# Autodesk Inventor assembly: PanelMountNew Sliced
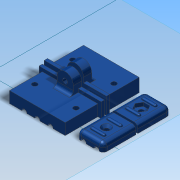
[picture p0: Inventor's stored thumbnail of the model, 180x180]
Saved by Autodesk Inventor 2014 SP2 (Build 180246200, 246)
## iProperties
Created: 2014-06-07
Part Number: PanelMountNew Sliced
Document SubType Name: Assembly
Designer: dliu
Author: dliu
## Documents named in this file (8)
- C:\Users\dliu\Dropbox\dbhome\electric-longboard\dliu\PanelMountNew Sliced.iam
- C:\Users\dliu\Dropbox\dbhome\electric-longboard\dliu\Electronics\Solid2.ipt
- C:\Users\dliu\Dropbox\dbhome\electric-longboard\dliu\Electronics\Solid3.ipt
- C:\Users\dliu\Dropbox\dbhome\electric-longboard\dliu\Electronics\Solid4.ipt
- C:\Users\dliu\Dropbox\dbhome\electric-longboard\dliu\Electronics\Solid5.ipt
- C:\Users\dliu\Dropbox\dbhome\electric-longboard\dliu\Electronics\Solid6.ipt
- C:\Users\dliu\Dropbox\dbhome\electric-longboard\dliu\Electronics\Solid7.ipt
- C:\Users\dliu\Dropbox\dbhome\electric-longboard\dliu\Electronics\Key.iam
## Components (7 placed, 7 different names)
1. Solid2:1 — Mate:5
2. Solid3:1 — Mate:4
3. Solid4:1 — Mate:3
4. Solid5:1 — Mate:2
5. Solid6:1 — Mate:1
6. Solid7:1 — Mate:6
7. Key:1 [sub-assembly] — Mate:7
## Relationships (7: Mate 7)
- Mate:1: Solid6:1
- Mate:2: Solid5:1
- Mate:3: Solid4:1
- Mate:4: Solid3:1
- Mate:5: Solid2:1
- Mate:6: Solid7:1
- Mate:7: Key:1
